# Autodesk Inventor assembly: Full payload assembly with plate
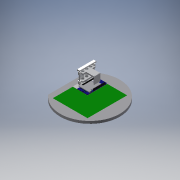
[picture p0: Inventor's stored thumbnail of the model, 180x180]
Saved by Autodesk Inventor 2017 (Build 210142000, 142)
## iProperties
Created: 2016-12-06
Part Number: Full payload assembly with plate
Document SubType Name: Assembly
Designer: qupec
Author: qupec
## Documents named in this file (2)
- C:\Users\qupec\Desktop\RockSat\Actual payload\New folder\Full payload assembly with plate.iam
- C:\Users\qupec\Desktop\RockSat\Actual payload\New folder\RockSat Plate.ipt
## Components (2 placed, 2 different names)
1. RockSat Plate:1 — Mate:1, Mate:2
2. Full payload assembly:1 [sub-assembly] — Mate:1, Mate:2
## Relationships (2: Mate 2)
- Mate:1: RockSat Plate:1 ↔ Full payload assembly:1
- Mate:2: RockSat Plate:1 ↔ Full payload assembly:1
